# Autodesk Inventor assembly: Montagem1
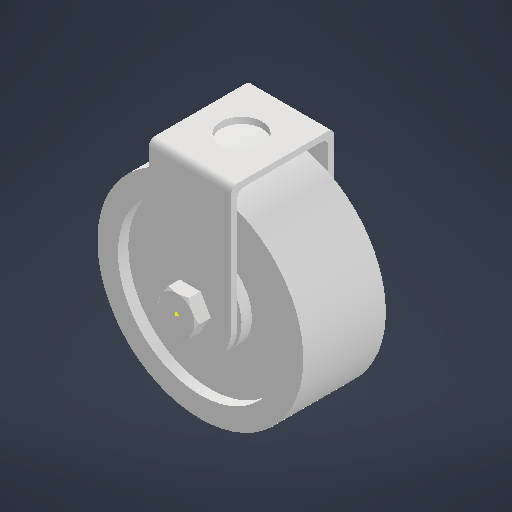
[picture p0: Inventor's stored thumbnail of the model, 512x512]
Saved by Autodesk Inventor 2027.1 (Build 311270010, 270A)
## iProperties
Created: 2026-08-27
Part Number: Montagem1
Document SubType Name: Assembly
Designer: labsfiap
Author: labsfiap
## Documents named in this file (7)
- C:\Users\labsfiap\Downloads\Trabalho_1\Montagem1.iam
- C:\Users\labsfiap\Downloads\Trabalho_1\6Peça_.ipt
- C:\Users\labsfiap\Downloads\Trabalho_1\5Peça_.ipt
- C:\Users\labsfiap\Downloads\Trabalho_1\4Peça_.ipt
- C:\Users\labsfiap\Downloads\Trabalho_1\3Peça_.ipt
- C:\Users\labsfiap\Downloads\Trabalho_1\2Peça_.ipt
- C:\Users\labsfiap\Downloads\Trabalho_1\1Peça_.ipt
## Components (7 placed, 6 different names)
1. 6Peça_:1 — Inserir:1, Inserir:2
2. 5Peça_:1 — Inserir:4
3. 4Peça_:1 — Inserir:5
4. 3Peça_:1 — Inserir:6
5. 2Peça_:1 — Inserir:2, Inserir:3, Inserir:4, Inserir:5, Inserir:6
6. 1Peça_:1 — Inserir:1
7. 5Peça_:2 — Inserir:3
## Relationships (6: Insert 6)
- Inserir:1: 6Peça_:1 ↔ 1Peça_:1
- Inserir:2 (2 mm): 6Peça_:1 ↔ 2Peça_:1
- Inserir:3: 2Peça_:1 ↔ 5Peça_:2
- Inserir:4: 5Peça_:1 ↔ 2Peça_:1
- Inserir:5 (-23 mm): 4Peça_:1 ↔ 2Peça_:1
- Inserir:6: 3Peça_:1 ↔ 2Peça_:1
